# Autodesk Inventor assembly: 200-20-ROCKER-CONNECTOR-ASM-01
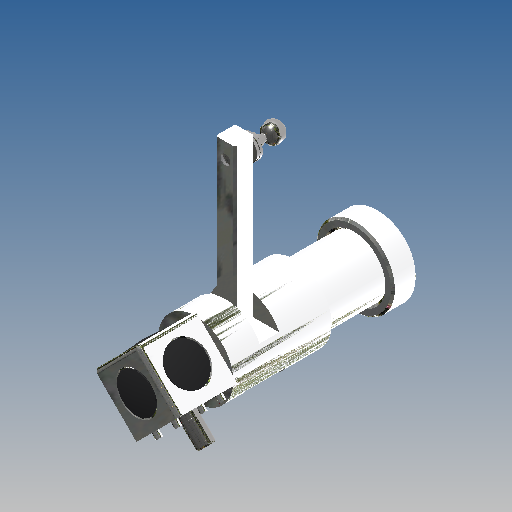
[picture p0: Inventor's stored thumbnail of the model, 512x512]
Saved by Autodesk Inventor 2018.2 (Build 222227000, 227)
## iProperties
Manager: feesmrt
Company: FRANC0R
Created: 2017-11-01
Part Number: 200-20-ROCKER-CONNECTOR-ASM-01
Material: Generisch
Document SubType Name: Assembly
Designer: feesmrt
Project: Rescue Robot
Cost Center: -
Description: Rocker Bearing Connector
Engineer: feesmrt
Authority: feesmrt
Stock Number: 200-20-ROCKER-CONNECTOR-ASM-01
Author: feesmrt
Title: Rocker Bearing Connector
Subject: Rescue Robot
Revision Number: 1
## Documents named in this file (8)
- D:\Programmierung\FRANC0R\CAD\02-Rocker-Bogie-Robot\200-ROCKER-BOGIE\200-20-ROCKER-CONNECTOR\200-20-ROCKER-CONNECTOR-ASM-01.iam
- D:\Programmierung\FRANC0R\CAD\02-Rocker-Bogie-Robot\200-ROCKER-BOGIE\200-20-ROCKER-CONNECTOR\200-20-ROCKER-CONNECTOR-01.ipt
- D:\Programmierung\FRANC0R\CAD\02-Rocker-Bogie-Robot\200-ROCKER-BOGIE\200-20-ROCKER-CONNECTOR\200-20-ROCKER-CONNECTOR-02.ipt
- D:\Programmierung\FRANC0R\CAD\02-Rocker-Bogie-Robot\900-COMPONENTS\900-40-SCREWS\900-40-SCREWS-ISO10642_M6x16.ipt
- D:\Programmierung\FRANC0R\CAD\02-Rocker-Bogie-Robot\900-COMPONENTS\900-50-PROFILES\90-50-PROFILES-QUAD-CONN-30x30.ipt
- D:\Programmierung\FRANC0R\CAD\02-Rocker-Bogie-Robot\900-COMPONENTS\900-50-PROFILES\90-50-PROFILES-QUAD-CONN-30x30-CAP.ipt
- D:\Programmierung\FRANC0R\CAD\02-Rocker-Bogie-Robot\900-COMPONENTS\900-40-SCREWS\900-40-SCREWS-ISO10642_M8x20.ipt
- D:\Programmierung\FRANC0R\CAD\02-Rocker-Bogie-Robot\200-ROCKER-BOGIE\200-60-DIFFERENTIAL\200-60-DIFFERENTIAL-BAR-01.iam
## Components (11 placed, 7 different names)
1. 200-20-ROCKER-CONNECTOR-01:1 — Passend:1, Passend:2, Passend:5, Passend:6, Passend:7, Passend:23, Passend:26, Passend:27, Passend:28
2. 200-20-ROCKER-CONNECTOR-02:1 — Passend:1, Passend:2, Passend:4, Fluchtend:1
3. 900-40-SCREWS-ISO10642_M6x16:1 — Passend:4, Fluchtend:1
4. 90-50-PROFILES-QUAD-CONN-30x30:1 — Passend:5, Passend:6, Passend:7, Passend:15, Passend:16, Passend:17, Passend:18, Passend:19, Passend:20, Passend:22, Fluchtend:24, Fluchtend:25, Fluchtend:26, Passend:24, Passend:25
5. 900-40-SCREWS-ISO10642_M8x20:1 — Passend:22, Fluchtend:24, Passend:24
6. 900-40-SCREWS-ISO10642_M8x20:2 — Passend:23, Fluchtend:26
7. 900-40-SCREWS-ISO10642_M8x20:3 — Fluchtend:25, Passend:25
8. 90-50-PROFILES-QUAD-CONN-30x30-CAP:2 — Passend:17, Passend:18
9. 90-50-PROFILES-QUAD-CONN-30x30-CAP:3 — Passend:15, Passend:16
10. 90-50-PROFILES-QUAD-CONN-30x30-CAP:4 — Passend:19, Passend:20
11. 200-60-DIFFERENTIAL-BAR-01:1 [sub-assembly] — Passend:26, Passend:27, Passend:28
## Relationships (23: Mate 19, Flush 4)
- Passend:1 [Mate]: 200-20-ROCKER-CONNECTOR-01:1 ↔ 200-20-ROCKER-CONNECTOR-02:1
- Passend:2 [Mate]: 200-20-ROCKER-CONNECTOR-01:1 ↔ 200-20-ROCKER-CONNECTOR-02:1
- Passend:4 [Mate]: 200-20-ROCKER-CONNECTOR-02:1 ↔ 900-40-SCREWS-ISO10642_M6x16:1
- Fluchtend:1 [Flush]: 200-20-ROCKER-CONNECTOR-02:1 ↔ 900-40-SCREWS-ISO10642_M6x16:1
- Passend:5 [Mate]: 200-20-ROCKER-CONNECTOR-01:1 ↔ 90-50-PROFILES-QUAD-CONN-30x30:1
- Passend:6 [Mate]: 200-20-ROCKER-CONNECTOR-01:1 ↔ 90-50-PROFILES-QUAD-CONN-30x30:1
- Passend:7 [Mate]: 200-20-ROCKER-CONNECTOR-01:1 ↔ 90-50-PROFILES-QUAD-CONN-30x30:1
- Passend:15 [Mate]: 90-50-PROFILES-QUAD-CONN-30x30:1 ↔ 90-50-PROFILES-QUAD-CONN-30x30-CAP:3
- Passend:16 [Mate]: 90-50-PROFILES-QUAD-CONN-30x30:1 ↔ 90-50-PROFILES-QUAD-CONN-30x30-CAP:3
- Passend:17 [Mate]: 90-50-PROFILES-QUAD-CONN-30x30:1 ↔ 90-50-PROFILES-QUAD-CONN-30x30-CAP:2
- Passend:18 [Mate]: 90-50-PROFILES-QUAD-CONN-30x30:1 ↔ 90-50-PROFILES-QUAD-CONN-30x30-CAP:2
- Passend:19 [Mate]: 90-50-PROFILES-QUAD-CONN-30x30:1 ↔ 90-50-PROFILES-QUAD-CONN-30x30-CAP:4
- Passend:20 [Mate]: 90-50-PROFILES-QUAD-CONN-30x30:1 ↔ 90-50-PROFILES-QUAD-CONN-30x30-CAP:4
- Passend:22 [Mate]: 90-50-PROFILES-QUAD-CONN-30x30:1 ↔ 900-40-SCREWS-ISO10642_M8x20:1
- Passend:23 [Mate]: 200-20-ROCKER-CONNECTOR-01:1 ↔ 900-40-SCREWS-ISO10642_M8x20:2
- Fluchtend:24 [Flush]: 90-50-PROFILES-QUAD-CONN-30x30:1 ↔ 900-40-SCREWS-ISO10642_M8x20:1
- Fluchtend:25 [Flush]: 90-50-PROFILES-QUAD-CONN-30x30:1 ↔ 900-40-SCREWS-ISO10642_M8x20:3
- Fluchtend:26 [Flush]: 90-50-PROFILES-QUAD-CONN-30x30:1 ↔ 900-40-SCREWS-ISO10642_M8x20:2
- Passend:24 [Mate]: 90-50-PROFILES-QUAD-CONN-30x30:1 ↔ 900-40-SCREWS-ISO10642_M8x20:1
- Passend:25 [Mate]: 90-50-PROFILES-QUAD-CONN-30x30:1 ↔ 900-40-SCREWS-ISO10642_M8x20:3
- Passend:26 [Mate]: 200-20-ROCKER-CONNECTOR-01:1 ↔ 200-60-DIFFERENTIAL-BAR-01:1
- Passend:27 [Mate]: 200-20-ROCKER-CONNECTOR-01:1 ↔ 200-60-DIFFERENTIAL-BAR-01:1
- Passend:28 [Mate]: 200-20-ROCKER-CONNECTOR-01:1 ↔ 200-60-DIFFERENTIAL-BAR-01:1
